# Autodesk Inventor assembly: Assembly2
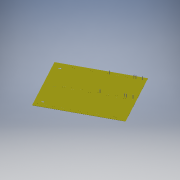
[picture p0: Inventor's stored thumbnail of the model, 180x180]
Saved by Autodesk Inventor 2019 (Build 230136000, 136)
## iProperties
Created: 2020-11-05
Part Number: Assembly2
Document SubType Name: Assembly
Designer: james
Author: james
## Documents named in this file (4)
- F:\JimsDesign\P1001-16bit-CPU\P1001-001 - 16bit CPU\P1001-001-004-320 - Register\Assembly2.iam
- F:\JimsDesign\P1001-16bit-CPU\P1001-001 - 16bit CPU\PRT1001-214 Base.ipt
- F:\JimsDesign\P1001-16bit-CPU\P1001-001 - 16bit CPU\P1001-001-004-320 - Register\Register.ipt
- F:\JimsDesign\P1001-16bit-CPU\P1001-001 - 16bit CPU\P1001-001-004-320 - Register\ALU.ipt
## Components (3 placed, 3 different names)
1. PRT1001-214 Base:1 — Mate:1, Mate:2, Mate:3, Mate:4, Mate:5, Mate:6
2. Register:1 — Mate:1, Mate:2, Mate:3
3. ALU:1 — Mate:4, Mate:5, Mate:6
## Relationships (6: Mate 6)
- Mate:1: PRT1001-214 Base:1 ↔ Register:1
- Mate:2: PRT1001-214 Base:1 ↔ Register:1
- Mate:3: PRT1001-214 Base:1 ↔ Register:1
- Mate:4: PRT1001-214 Base:1 ↔ ALU:1
- Mate:5: PRT1001-214 Base:1 ↔ ALU:1
- Mate:6: PRT1001-214 Base:1 ↔ ALU:1
